# Autodesk Inventor assembly: Mechanism Final
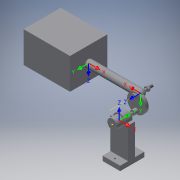
[picture p0: Inventor's stored thumbnail of the model, 180x180]
Saved by Autodesk Inventor 2019 (Build 230136000, 136)
## iProperties
Created: 2019-10-15
Part Number: Mechanism Final
Document SubType Name: Assembly
Designer: sudhanva
Author: sudhanva
## Documents named in this file (5)
- E:\Engineering softwares\3D Design\Mechanism Final.iam
- E:\Engineering softwares\3D Design\Piston Model.ipt
- E:\Engineering softwares\3D Design\AssemblyFinal.iam
- E:\Engineering softwares\3D Design\Nut.ipt
- E:\Engineering softwares\3D Design\Bolt.ipt
## Components (4 placed, 4 different names)
1. Piston Model:1 — Rigid:1, Cylindrical:1
2. AssemblyFinal:1 [sub-assembly] — Mate:1, Rigid:1
3. Nut:1 — Cylindrical:1, Rotational:1
4. Bolt:1 — Rotational:1
## Relationships (4: Mate 1, WeldJoint 1, CylindricalJoint 1, RevoluteJoint 1)
- Mate:1: AssemblyFinal:1
- Rigid:1 [WeldJoint]: Piston Model:1 ↔ AssemblyFinal:1
- Cylindrical:1: Piston Model:1 ↔ Nut:1
- Rotational:1 [RevoluteJoint] (-13.7 mm): Nut:1 ↔ Bolt:1
